# Autodesk Inventor assembly: 가스벨브 조립품
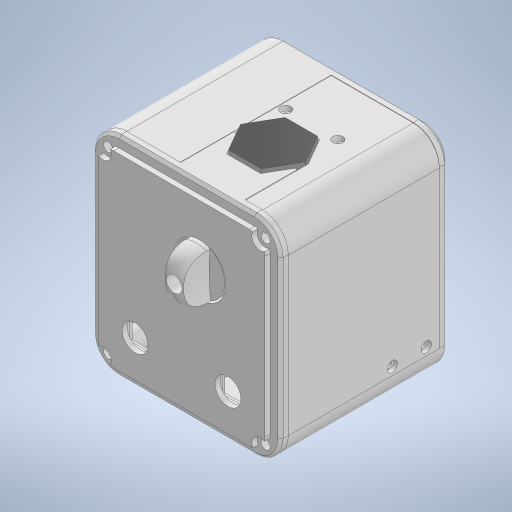
[picture p0: Inventor's stored thumbnail of the model, 512x512]
Saved by Autodesk Inventor 2023 (Build 270158000, 158)
## iProperties
Created: 2022-08-14
Part Number: 가스벨브 조립품
Document SubType Name: Assembly
Designer: fly01
Author: fly01
## Documents named in this file (12)
- C:\Users\user\Desktop\PAI\IOT부품\가스벨브\가스벨브 조립품.iam
- C:\Users\user\Desktop\PAI\IOT부품\가스벨브\가스벨브 기어.ipt
- C:\Users\user\Desktop\PAI\IOT부품\가스벨브\가스벨브 역설계.ipt
- C:\Users\user\Desktop\PAI\IOT부품\가스벨브\MG995서보모터.ipt
- C:\Users\user\Desktop\PAI\IOT부품\가스벨브\MG서보모터 원형부품.ipt
- C:\Users\user\Desktop\PAI\IOT부품\가스벨브\스텝모터 기어설계.ipt
- C:\Users\user\Desktop\PAI\IOT부품\esp32f.ipt
- C:\Users\user\Desktop\PAI\IOT부품\가스벨브\가스벨브 하우징.ipt
- C:\Users\user\Desktop\PAI\IOT부품\가스벨브\배터리 커버.ipt
- C:\Users\user\Desktop\PAI\IOT부품\가스벨브\가스벨브 하우징 커버.ipt
- C:\Users\user\Desktop\PAI\IOT부품\가스벨브\카스벨브 하단 커버.ipt
- C:\Users\user\Desktop\PAI\IOT부품\가스벨브\가스벨브 상단 커버.ipt
## Components (11 placed, 11 different names)
1. 가스벨브 기어:1 — 삽입:1
2. 가스벨브 역설계:1 — 삽입:1, 삽입:5, 각도:1
3. MG995서보모터:1 — 삽입:4, 삽입:6, 삽입:7
4. MG서보모터 원형부품:1 — 삽입:2, 삽입:3, 삽입:4
5. 스텝모터 기어설계:1 — 삽입:2, 삽입:3
6. esp32f:1 — 삽입:8, 삽입:9
7. 가스벨브 하우징:1 — 삽입:5, 삽입:6, 삽입:7, 삽입:8, 삽입:9, 각도:1, 삽입:12, 삽입:13, 삽입:14, 삽입:15, 삽입:17, 삽입:18, 삽입:19
8. 배터리 커버:1 — 삽입:19
9. 가스벨브 하우징 커버:1 — 삽입:12, 삽입:13
10. 카스벨브 하단 커버:1 — 삽입:14, 삽입:15
11. 가스벨브 상단 커버:1 — 삽입:17, 삽입:18
## Relationships (17: Insert 16, Angle 1)
- 삽입:1 [Insert]: 가스벨브 기어:1 ↔ 가스벨브 역설계:1
- 삽입:2 [Insert]: MG서보모터 원형부품:1 ↔ 스텝모터 기어설계:1
- 삽입:3 [Insert]: MG서보모터 원형부품:1 ↔ 스텝모터 기어설계:1
- 삽입:4 [Insert]: MG995서보모터:1 ↔ MG서보모터 원형부품:1
- 삽입:5 [Insert]: 가스벨브 역설계:1 ↔ 가스벨브 하우징:1
- 삽입:6 [Insert]: MG995서보모터:1 ↔ 가스벨브 하우징:1
- 삽입:7 [Insert]: MG995서보모터:1 ↔ 가스벨브 하우징:1
- 삽입:8 [Insert]: esp32f:1 ↔ 가스벨브 하우징:1
- 삽입:9 [Insert]: esp32f:1 ↔ 가스벨브 하우징:1
- 각도:1 [Angle] (0 deg): 가스벨브 역설계:1 ↔ 가스벨브 하우징:1
- 삽입:12 [Insert]: 가스벨브 하우징:1 ↔ 가스벨브 하우징 커버:1
- 삽입:13 [Insert]: 가스벨브 하우징:1 ↔ 가스벨브 하우징 커버:1
- 삽입:14 [Insert]: 가스벨브 하우징:1 ↔ 카스벨브 하단 커버:1
- 삽입:15 [Insert]: 가스벨브 하우징:1 ↔ 카스벨브 하단 커버:1
- 삽입:17 [Insert]: 가스벨브 하우징:1 ↔ 가스벨브 상단 커버:1
- 삽입:18 [Insert]: 가스벨브 하우징:1 ↔ 가스벨브 상단 커버:1
- 삽입:19 [Insert]: 가스벨브 하우징:1 ↔ 배터리 커버:1
